# Autodesk Inventor assembly: Assembly_Cube_Alignment_Tool_with_Pinhole
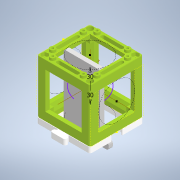
[picture p0: Inventor's stored thumbnail of the model, 180x180]
Saved by Autodesk Inventor 2022.3 (Build 263350000, 350)
## iProperties
Created: 2022-07-22
Part Number: Assembly_Cube_Alignment_Tool_with_Pinhole
Document SubType Name: Assembly
Designer: bingoeleda
Author: bingoeleda
## Documents named in this file (3)
- G:\My Drive\ASP - M.Sc. Photonics\Practical Modules\MODULE 4 - Master Thesis\2.Experiments\Modules\15.Alignment Tool\Assembly_Cube_Alignment_Tool_with_Pinhole.iam
- G:\My Drive\ASP - M.Sc. Photonics\Practical Modules\MODULE 4 - Master Thesis\2.Experiments\Modules\2.Base_Cube\Base_Cube_IM\Assembly_Cube_empty_IM_withBase_v3.iam
- G:\My Drive\ASP - M.Sc. Photonics\Practical Modules\MODULE 4 - Master Thesis\2.Experiments\Modules\15.Alignment Tool\00_Slider_Mask_Darkfield.ipt
## Components (2 placed, 2 different names)
1. Assembly_Cube_empty_IM_withBase_v3:1 [sub-assembly] — Mate:1, Mate:2, Mate:3, Mate:4, Mate:5, Mate:6, Mate:7
2. 00_Slider_Mask_Darkfield:1 — Mate:1, Mate:2, Mate:3, Mate:4, Mate:5, Mate:7
## Relationships (7: Mate 7)
- Mate:1: Assembly_Cube_empty_IM_withBase_v3:1 ↔ 00_Slider_Mask_Darkfield:1
- Mate:2: Assembly_Cube_empty_IM_withBase_v3:1 ↔ 00_Slider_Mask_Darkfield:1
- Mate:3: Assembly_Cube_empty_IM_withBase_v3:1 ↔ 00_Slider_Mask_Darkfield:1
- Mate:4: Assembly_Cube_empty_IM_withBase_v3:1 ↔ 00_Slider_Mask_Darkfield:1
- Mate:5: Assembly_Cube_empty_IM_withBase_v3:1 ↔ 00_Slider_Mask_Darkfield:1
- Mate:6: Assembly_Cube_empty_IM_withBase_v3:1
- Mate:7: Assembly_Cube_empty_IM_withBase_v3:1 ↔ 00_Slider_Mask_Darkfield:1
